# Autodesk Inventor assembly: stepperGearBoxSystemTilt
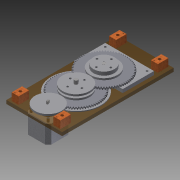
[picture p0: Inventor's stored thumbnail of the model, 180x180]
Saved by Autodesk Inventor 2013 (Build 170138000, 138)
## iProperties
Created: 2014-07-03
Part Number: stepperGearBoxSystemTilt
Document SubType Name: Assembly
Designer: Nano
Author: Nano
## Documents named in this file (11)
- C:\Users\Nano\Documents\InventorByron\InventorMasterProject\panTiltSystem\stepperGearBoxSystemTilt.iam
- C:\Users\Nano\Documents\InventorByron\InventorMasterProject\panTiltSystem\stepper42BYGH007_RB01.ipt
- C:\Users\Nano\Documents\InventorByron\InventorMasterProject\panTiltSystem\gearExperiments\gearTry01.iam
- C:\Users\Nano\Documents\InventorByron\InventorMasterProject\panTiltSystem\panGearShaft1.ipt
- C:\Users\Nano\Documents\InventorByron\InventorMasterProject\panTiltSystem\panGearSpacerBlocks.ipt
- C:\Users\Nano\Documents\InventorByron\InventorMasterProject\panTiltSystem\gearSpacerDisc01.ipt
- C:\Users\Nano\Documents\InventorByron\InventorMasterProject\panTiltSystem\gearGuideDiscOutputStage1.ipt
- C:\Users\Nano\Documents\InventorByron\InventorMasterProject\panTiltSystem\gearSpacerSmallOutputStage.ipt
- C:\Users\Nano\Documents\InventorByron\InventorMasterProject\panTiltSystem\panTilt_RB02_cutFiles\cutFiles125\driveGearCap.ipt
- C:\Users\Nano\Documents\InventorByron\InventorMasterProject\panTiltSystem\panTilt_RB02_cutFiles\cutFiles125\outputGearSupport.ipt
- C:\Users\Nano\Documents\InventorByron\InventorMasterProject\panTiltSystem\panTilt_RB02_cutFiles\cutFiles25\driveGearSupportLayer.ipt
## Components (17 placed, 10 different names)
1. stepper42BYGH007_RB01:1
2. gearTry01:1 [sub-assembly]
3. panGearShaft1:1
4. panGearSpacerBlocks:1
5. panGearSpacerBlocks:2
6. panGearSpacerBlocks:3
7. panGearSpacerBlocks:4
8. gearSpacerDisc01:1
9. gearSpacerDisc01:2
10. gearGuideDiscOutputStage1:1
11. gearSpacerDisc01:3
12. gearSpacerDisc01:4
13. gearSpacerSmallOutputStage:1
14. panGearShaft1:2
15. driveGearCap:1
16. outputGearSupport:1
17. driveGearSupportLayer:1
## Relationships (31: Mate 14, Flush 14, Angle 3)
- [Mate]: stepper42BYGH007_RB01:1 ↔ gearTry01:1
- [Mate]: stepper42BYGH007_RB01:1 ↔ gearTry01:1
- [Flush]: gearTry01:1 ↔ panGearShaft1:1
- [Flush]: gearTry01:1 ↔ panGearShaft1:1
- [Flush]: gearTry01:1 ↔ panGearSpacerBlocks:1
- [Flush]: gearTry01:1 ↔ panGearSpacerBlocks:1
- [Mate]: gearTry01:1 ↔ panGearSpacerBlocks:2
- [Mate]: gearTry01:1 ↔ panGearSpacerBlocks:2
- [Angle] (0 deg): gearTry01:1 ↔ panGearSpacerBlocks:2
- [Mate]: gearTry01:1 ↔ panGearSpacerBlocks:3
- [Mate]: gearTry01:1 ↔ panGearSpacerBlocks:3
- [Angle] (0 deg): gearTry01:1 ↔ panGearSpacerBlocks:3
- [Mate]: gearTry01:1 ↔ panGearSpacerBlocks:4
- [Mate]: gearTry01:1 ↔ panGearSpacerBlocks:4
- [Angle] (0 deg): gearTry01:1 ↔ panGearSpacerBlocks:4
- [Flush]: gearTry01:1 ↔ gearSpacerDisc01:1
- [Flush]: gearTry01:1 ↔ gearSpacerDisc01:1
- [Mate]: panGearShaft1:1 ↔ gearSpacerDisc01:2
- [Mate]: gearGuideDiscOutputStage1:1 ↔ gearSpacerDisc01:3
- [Mate]: gearTry01:1 ↔ gearSpacerDisc01:3
- [Mate]: gearTry01:1 ↔ gearSpacerDisc01:4
- [Mate]: gearTry01:1 ↔ gearSpacerDisc01:4
- [Flush]: gearSpacerDisc01:4 ↔ gearSpacerSmallOutputStage:1
- [Flush]: gearSpacerDisc01:4 ↔ gearSpacerSmallOutputStage:1
- [Mate]: gearTry01:1 ↔ panGearShaft1:2
- [Flush]: gearTry01:1 ↔ panGearShaft1:2
- [Flush]: gearTry01:1 ↔ driveGearCap:1
- [Flush]: gearTry01:1 ↔ outputGearSupport:1
- [Flush]: gearTry01:1 ↔ outputGearSupport:1
- [Flush]: gearTry01:1 ↔ driveGearSupportLayer:1
- [Flush]: gearTry01:1 ↔ driveGearSupportLayer:1
